# Autodesk Inventor assembly: top_shaft_mirrored
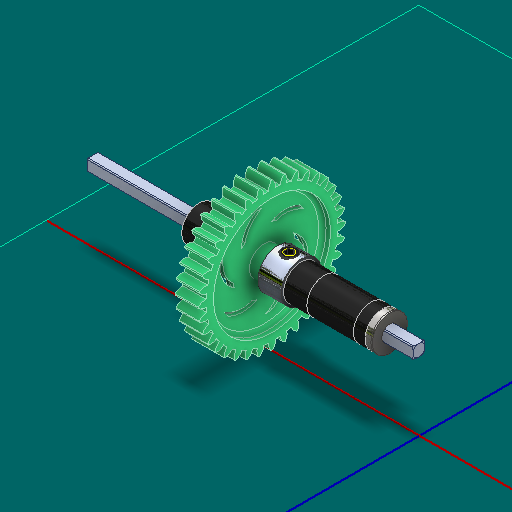
[picture p0: Inventor's stored thumbnail of the model, 512x512]
Saved by Autodesk Inventor 2025 (Build 290162000, 162)
## iProperties
Created: 2024-08-16
Part Number: top_shaft_mirrored
Document SubType Name: Assembly
Designer: averey
Author: averey
## Documents named in this file (14)
- C:\Users\avere\vex_robotics_high_stakes\hardware\cad\ATLAS\chassis\drive_pod\back_left\gearbox\top_shaft_mirrored.iam
- C:\Users\avere\vex_robotics_high_stakes\hardware\cad\VEX-CAD-Inventor\Motion\Shaft LS\Shaft LS\Shaft LS 3.5.ipt
- C:\Users\avere\vex_robotics_high_stakes\hardware\cad\VEX-CAD-Inventor\Motion\Shaft LS\Shaft LS.ipt
- C:\Users\avere\vex_robotics_high_stakes\hardware\cad\ATLAS\chassis\drive_pod\back_left\gearbox\LS 36T Gear_mirrored.ipt
- C:\Users\avere\vex_robotics_high_stakes\hardware\cad\VEX-CAD-Inventor\Motion\Spacers\Spacer Nylon .375 OD\NSpacer .375 OD x .375.ipt
- C:\Users\avere\vex_robotics_high_stakes\hardware\cad\VEX-CAD-Inventor\Motion\Spacers\Spacer Nylon .375 OD.ipt
- C:\Users\avere\vex_robotics_high_stakes\hardware\cad\VEX-CAD-Inventor\Motion\Spacers\Washer Steel\SWasher .375 OD x .062500.ipt
- C:\Users\avere\vex_robotics_high_stakes\hardware\cad\VEX-CAD-Inventor\Motion\Spacers\Washer Steel.ipt
- C:\Users\avere\vex_robotics_high_stakes\hardware\cad\VEX-CAD-Inventor\Motion\Spacers\Washer Steel\SWasher .375 OD x .015625.ipt
- C:\Users\avere\vex_robotics_high_stakes\hardware\cad\VEX-CAD-Inventor\Motion\Spacers\Spacer Nylon .375 OD\NSpacer .375 OD x .125.ipt
- C:\Users\avere\vex_robotics_high_stakes\hardware\cad\VEX-CAD-Inventor\Motion\Spacers\Spacer Nylon .375 OD\NSpacer .375 OD x .500.ipt
- C:\Users\avere\vex_robotics_high_stakes\hardware\cad\VEX-CAD-Inventor\Motion\Spacers\Spacer Nylon .375 OD\NSpacer .375 OD x .250.ipt
- C:\Users\avere\vex_robotics_high_stakes\hardware\cad\ATLAS\chassis\drive_pod\back_left\gearbox\Shaft Collar Set Screw_mirrored.ipt
- C:\Users\avere\vex_robotics_high_stakes\hardware\cad\VEX-CAD-Inventor\Motion\Spacers\Washer Steel\SWasher .375 OD x .031250.ipt
## Components (11 placed, 10 different names)
1. Shaft LS 3.5:1 — Mate:1, Insert:1, Angle:1
2. LS 36T Gear_mirrored:1 — Insert:1, Angle:1, Insert:3, Insert:10
3. NSpacer .375 OD x .375:1 — Insert:15
4. SWasher .375 OD x .062500:1 — Insert:3, Insert:14
5. SWasher .375 OD x .015625:2 — Insert:13
6. SWasher .375 OD x .062500:3 — Insert:13, Insert:9
7. NSpacer .375 OD x .125:2 — Insert:9, Insert:6
8. NSpacer .375 OD x .500:3 — Insert:6, Insert:12
9. NSpacer .375 OD x .250:4 — Insert:12, Insert:11
10. Shaft Collar Set Screw_mirrored:1 — Insert:11, Insert:10
11. SWasher .375 OD x .031250:4 — Insert:15, Insert:14
## Relationships (12: Insert 10, Mate 1, Angle 1)
- Mate:1: Shaft LS 3.5:1
- Insert:1 (38.4969 mm): Shaft LS 3.5:1 ↔ LS 36T Gear_mirrored:1
- Angle:1 (0 deg): Shaft LS 3.5:1 ↔ LS 36T Gear_mirrored:1
- Insert:3: LS 36T Gear_mirrored:1 ↔ SWasher .375 OD x .062500:1
- Insert:13: SWasher .375 OD x .015625:2 ↔ SWasher .375 OD x .062500:3
- Insert:9: SWasher .375 OD x .062500:3 ↔ NSpacer .375 OD x .125:2
- Insert:6: NSpacer .375 OD x .125:2 ↔ NSpacer .375 OD x .500:3
- Insert:12: NSpacer .375 OD x .500:3 ↔ NSpacer .375 OD x .250:4
- Insert:11: NSpacer .375 OD x .250:4 ↔ Shaft Collar Set Screw_mirrored:1
- Insert:10: LS 36T Gear_mirrored:1 ↔ Shaft Collar Set Screw_mirrored:1
- Insert:15: NSpacer .375 OD x .375:1 ↔ SWasher .375 OD x .031250:4
- Insert:14: SWasher .375 OD x .062500:1 ↔ SWasher .375 OD x .031250:4
